# Autodesk Inventor assembly: Contrapeso
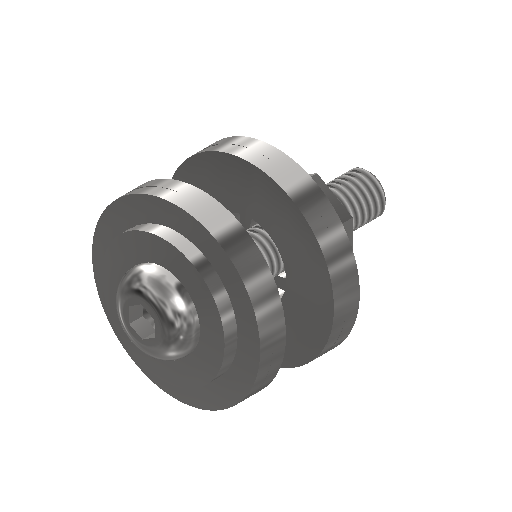
[picture p0: Inventor's stored thumbnail of the model, 512x512]
Saved by Autodesk Inventor 2025.3 (Build 293356000, 356)
## iProperties
Created: 2025-11-11
Part Number: Contrapeso
Document SubType Name: Assembly
Designer: Gabriel Bojaca
Mass: 5.85443 g
Surface Area: 17.43 cm^2
Volume: 0.734492 cm^3
Density: 7.97072 g/cm^3
Author: Gabriel Bojaca
## Documents named in this file (5)
- C:\Users\Gabriel Bojaca\Documents\Inventor\TDC\Contrapeso.iam
- C:\Users\Gabriel Bojaca\Documents\Inventor\Content Center Files\R2025\en-US\ANSI B18.3.4M(1)\ANSI B18.3.4M - M3 x 0.5 x 16(2).ipt
- C:\Users\Gabriel Bojaca\Documents\Inventor\TDC\Arandela_3_16.ipt
- C:\Users\Gabriel Bojaca\Documents\Inventor\TDC\Arandela_1_8.ipt
- C:\Users\Gabriel Bojaca\Documents\Inventor\TDC\Tuerca_M3.ipt
## Components (8 placed, 4 different names)
1. Broached Hexagon Socket Button Head Cap Screw - Metric M3 x 0.5 x 16:3 — Mate:88, Mate:89, Mate:91, Mate:93, Mate:97, Mate:98, Mate:101, Mate:102
2. Arandela_3_16:1 — Mate:97, Mate:99
3. Arandela_1_8:1 — Mate:100, Mate:101, Mate:103
4. Arandela_3_16:2 — Mate:89, Mate:90, Mate:92
5. Arandela_1_8:2 — Mate:88, Mate:90, Mate:91
6. Tuerca_M3:2 — Mate:102, Mate:103
7. Arandela_3_16:3 — Mate:98, Mate:99, Mate:100
8. Arandela_3_16:4 — Mate:92, Mate:93
## Relationships (13: Mate 13)
- Mate:88: Broached Hexagon Socket Button Head Cap Screw - Metric M3 x 0.5 x 16:3 ↔ Arandela_1_8:2
- Mate:89: Broached Hexagon Socket Button Head Cap Screw - Metric M3 x 0.5 x 16:3 ↔ Arandela_3_16:2
- Mate:90: Arandela_3_16:2 ↔ Arandela_1_8:2
- Mate:91: Broached Hexagon Socket Button Head Cap Screw - Metric M3 x 0.5 x 16:3 ↔ Arandela_1_8:2
- Mate:92: Arandela_3_16:2 ↔ Arandela_3_16:4
- Mate:93: Broached Hexagon Socket Button Head Cap Screw - Metric M3 x 0.5 x 16:3 ↔ Arandela_3_16:4
- Mate:97: Broached Hexagon Socket Button Head Cap Screw - Metric M3 x 0.5 x 16:3 ↔ Arandela_3_16:1
- Mate:98: Broached Hexagon Socket Button Head Cap Screw - Metric M3 x 0.5 x 16:3 ↔ Arandela_3_16:3
- Mate:99: Arandela_3_16:1 ↔ Arandela_3_16:3
- Mate:100: Arandela_1_8:1 ↔ Arandela_3_16:3
- Mate:101: Broached Hexagon Socket Button Head Cap Screw - Metric M3 x 0.5 x 16:3 ↔ Arandela_1_8:1
- Mate:102: Broached Hexagon Socket Button Head Cap Screw - Metric M3 x 0.5 x 16:3 ↔ Tuerca_M3:2
- Mate:103: Arandela_1_8:1 ↔ Tuerca_M3:2
